# Autodesk Inventor assembly: КВ33-AN1-01-00-Колесо
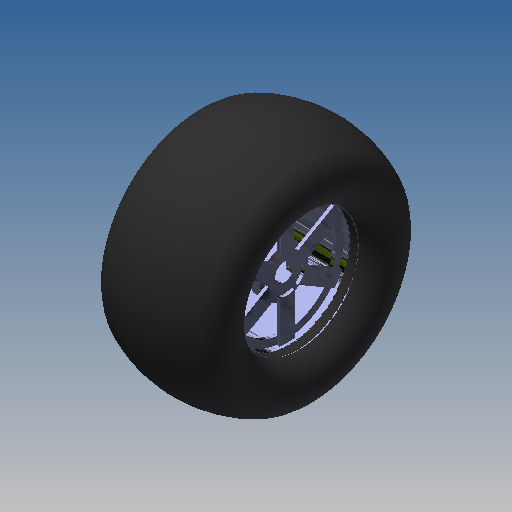
[picture p0: Inventor's stored thumbnail of the model, 512x512]
Saved by Autodesk Inventor 2020 (Build 240168000, 168)
## iProperties
Part Number: КВ33-AN1-01-00-Колесо
Material: Типовые
Document SubType Name: Assembly
Designer: sbnnl
Mass: 1000.36 g
Surface Area: 1140.53 cm^2
Volume: 1000.36 cm^3
Density: 1 g/cm^3
Author: sbnnl
## Documents named in this file (3)
- E:\IVAN\Ivan_desktop\Kvantorium\Projects\RoboPatrol\design\standart_components\WheelBig\колесо большое.iam
- E:\IVAN\Ivan_desktop\Kvantorium\Projects\RoboPatrol\design\standart_components\WheelBig\диск.ipt
- E:\IVAN\Ivan_desktop\Kvantorium\Projects\RoboPatrol\design\standart_components\WheelBig\шина.ipt
## Components (2 placed, 2 different names)
1. шина:1 — Совмещение:1
2. диск:1 — Совмещение:1
## Relationships (1: Mate 1)
- Совмещение:1 [Mate]: шина:1 ↔ диск:1
